# Autodesk Inventor assembly: TAKEONE 3D Printer
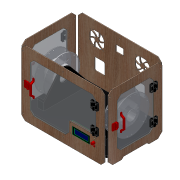
[picture p0: Inventor's stored thumbnail of the model, 180x180]
Saved by Autodesk Inventor 2015 (Build 190159000, 159)
## iProperties
Created: 2018-04-12
Part Number: TAKEONE 3D Printer
Document SubType Name: Assembly
Designer: Ghassan Yusuf
Author: Ghassan Yusuf
## Documents named in this file (14)
- X:\TAKEONE\Products\takeone-3D-printer\model\3D\TAKEONE 3D Printer.iam
- X:\TAKEONE\Products\takeone-3D-printer\model\3D\Front Face.ipt
- X:\TAKEONE\Products\takeone-3D-printer\model\3D\BackCover.ipt
- X:\TAKEONE\Products\takeone-3D-printer\model\3D\Left Sides Cover.ipt
- X:\TAKEONE\Products\takeone-3D-printer\model\3D\Right Sides Cover.ipt
- X:\TAKEONE\Products\takeone-3D-printer\model\3D\Front Clear Door Assambly.iam
- X:\TAKEONE\Products\takeone-3D-printer\model\3D\printer floor plate.ipt
- X:\TAKEONE\Products\takeone-3D-printer\model\3D\Spool Unit.iam
- X:\TAKEONE\Products\takeone-3D-printer\model\3D\Right Door Assembly.iam
- X:\TAKEONE\Products\takeone-3D-printer\model\3D\Left Door Assembly.iam
- X:\TAKEONE\Products\takeone-3D-printer\model\3D\2004A LCD Module.ipt
- X:\TAKEONE\Products\takeone-3D-printer\model\3D\Encoder Knobe.ipt
- X:\TAKEONE\Products\takeone-3D-printer\model\3D\Door Locks.ipt
- X:\TAKEONE\Products\takeone-3D-printer\model\3D\ResetButton.ipt
## Components (16 placed, 14 different names)
1. printer floor plate:1 — Mate:28, Flush:20, Mate:30, Mate:31, Mate:32, Flush:21, Flush:22, Flush:23, Mate:38
2. Door Locks:1 — Insert:12, Insert:13
3. Door Locks:2 — Insert:16, Insert:17
4. Door Locks:3 — Insert:14, Insert:15
5. Right Sides Cover:1 — Flush:14, Flush:15, Flush:16, Mate:30, Insert:9, Insert:10, Insert:16, Insert:17
6. Left Sides Cover:1 — Flush:11, Flush:12, Flush:13, Mate:28, Flush:20, Insert:7, Insert:8, Insert:14, Insert:15
7. Back Cover — Flush:5, Flush:7, Flush:10, Flush:13, Flush:16
8. Front Face — Flush:5, Flush:6, Mate:9, Flush:10, Flush:11, Flush:12, Flush:14, Flush:15, Insert:5, Insert:6, Mate:38, Flush:29, Mate:39, Mate:40, Insert:12, Insert:13, Insert:24
9. Left - Door Unit [sub-assembly] — Insert:9, Insert:10
10. Right - Door Unit [sub-assembly] — Insert:7, Insert:8
11. Front - Door Unit [sub-assembly] — Insert:5, Insert:6
12. Right - Spool Unit [sub-assembly] — Mate:32, Flush:22, Mate:33
13. Left - Spool Unit [sub-assembly] — Mate:31, Flush:21, Mate:33, Flush:23
14. Encoder Knobe:1 — Insert:11
15. 2004A LCD Module:1 — Insert:11, Flush:29, Mate:39, Mate:40
16. ResetButton:1 — Insert:24
## Relationships (38: Flush 15, Insert 14, Mate 9)
- Flush:5: Back Cover ↔ Front Face
- Flush:6: Front Face
- Flush:7: Back Cover
- Mate:9: Front Face
- Flush:10: Back Cover ↔ Front Face
- Flush:11: Left Sides Cover:1 ↔ Front Face
- Flush:12 (10 mm): Left Sides Cover:1 ↔ Front Face
- Flush:13 (10 mm): Left Sides Cover:1 ↔ Back Cover
- Flush:14: Right Sides Cover:1 ↔ Front Face
- Flush:15 (10 mm): Right Sides Cover:1 ↔ Front Face
- Flush:16 (10 mm): Right Sides Cover:1 ↔ Back Cover
- Mate:28: printer floor plate:1 ↔ Left Sides Cover:1
- Flush:20 (-8.7 mm): printer floor plate:1 ↔ Left Sides Cover:1
- Mate:30: printer floor plate:1 ↔ Right Sides Cover:1
- Mate:31: printer floor plate:1 ↔ Left - Spool Unit
- Mate:32: printer floor plate:1 ↔ Right - Spool Unit
- Flush:21 (80 mm): printer floor plate:1 ↔ Left - Spool Unit
- Flush:22 (80 mm): printer floor plate:1 ↔ Right - Spool Unit
- Mate:33: Right - Spool Unit ↔ Left - Spool Unit
- Flush:23: printer floor plate:1 ↔ Left - Spool Unit
- Insert:5: Front Face ↔ Front - Door Unit
- Insert:6: Front Face ↔ Front - Door Unit
- Mate:38: printer floor plate:1 ↔ Front Face
- Insert:7: Left Sides Cover:1 ↔ Right - Door Unit
- Insert:8: Left Sides Cover:1 ↔ Right - Door Unit
- Insert:9: Right Sides Cover:1 ↔ Left - Door Unit
- Insert:10: Right Sides Cover:1 ↔ Left - Door Unit
- Insert:11: Encoder Knobe:1 ↔ 2004A LCD Module:1
- Flush:29: Front Face ↔ 2004A LCD Module:1
- Mate:39 (0.3 mm): Front Face ↔ 2004A LCD Module:1
- Mate:40 (0.3 mm): Front Face ↔ 2004A LCD Module:1
- Insert:12: Door Locks:1 ↔ Front Face
- Insert:13: Door Locks:1 ↔ Front Face
- Insert:14: Door Locks:3 ↔ Left Sides Cover:1
- Insert:15: Door Locks:3 ↔ Left Sides Cover:1
- Insert:16: Door Locks:2 ↔ Right Sides Cover:1
- Insert:17: Door Locks:2 ↔ Right Sides Cover:1
- Insert:24: Front Face ↔ ResetButton:1
